# Autodesk Inventor assembly: assembled-feed
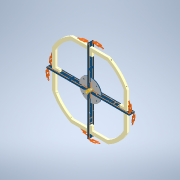
[picture p0: Inventor's stored thumbnail of the model, 180x180]
Saved by Autodesk Inventor 2021 (Build 250183000, 183)
## iProperties
Created: 2020-09-03
Part Number: assembled-feed
Document SubType Name: Assembly
Designer: dsouthall
Author: dsouthall
## iProperties of the stored document quad-slot-hub-traces.ipt
Created: 2020-10-19
Part Number: quad-slot-hub-traces
Material: Generic
Description: FreeCAD Model
Document SubType Name: Modeling
Designer: dsouthall
Authority: Unknown
Density: 1 g/cm^3
Appearance: Default
Sending System: FreeCAD
Preprocessor: Open CASCADE STEP processor 7.3
Title: C:/Users/dsouthall/OneDrive - The University of Chicago/Hpol/hpol-prototype/design/Feed Design/quad-slot-hub_revA/quad-slot-hub_revA/quad-slot-hub-traces.step
Author: Author
## iProperties of the stored document 91841A003_TYPE 18-8 STAINLESS STEEL HEX NUT.ipt
Created: 2015-02-23
Part Number: 91841A003_TYPE 18-8 STAINLESS STEEL HEX NUT
Material: Generic
Description: STEP AP203
Document SubType Name: Modeling
Designer: dsouthall
Density: 1 g/cm^3
Appearance: Default
Sending System: SolidWorks 2010
Preprocessor: SwSTEP 2.0
Title: 91841A003.step
Revision Number: ANY
## Documents named in this file (11)
- C:\Users\dsouthall\OneDrive - The University of Chicago\Hpol\hpol-prototype\design\Quad-Slot\Model 8 in\assembled-feed.iam
- C:\Users\dsouthall\OneDrive - The University of Chicago\Hpol\hpol-prototype\design\Quad-Slot\Model 8 in\assembled-feed_feedline_8in.iam
- C:\Users\dsouthall\OneDrive - The University of Chicago\Hpol\hpol-prototype\design\Quad-Slot\Model 8 in\source\standin_quad_hub.ipt
- C:\Users\dsouthall\OneDrive - The University of Chicago\Hpol\hpol-prototype\design\Quad-Slot\Model 8 in\source\insert_8in.ipt
- C:\Users\dsouthall\OneDrive - The University of Chicago\Hpol\hpol-prototype\design\Quad-Slot\Model 8 in\source\hub\COMPOUND.ipt
- **C:\Users\dsouthall\OneDrive - The University of Chicago\Hpol\hpol-prototype\design\Quad-Slot\Model 8 in\assembled-feed.iam*LocalDocs*xAaaaqbdaAaaaaaaaAaaaqho5Nc*quad-slot-hub-traces.ipt
- **C:\Users\dsouthall\OneDrive - The University of Chicago\Hpol\hpol-prototype\design\Quad-Slot\Model 8 in\assembled-feed.iam*LocalDocs*xAaaaqibaAaaaaaaaAaaaqomz3g*91841A003_TYPE 18-8 STAINLESS STEEL HEX NUT.ipt
- C:\Users\dsouthall\OneDrive - The University of Chicago\Hpol\hpol-prototype\design\Quad-Slot\Model 8 in\92196A077_18-8 STAINLESS STEEL SOCKET HEAD SCR.ipt
- C:\Users\dsouthall\OneDrive - The University of Chicago\Hpol\hpol-prototype\design\Feed Design\quad-slot-hub_revA\quad-slot-hub_revA\quad-slot-hub-traces.step
- C:\Users\dsouthall\OneDrive - The University of Chicago\Hpol\hpol-prototype\design\Quad-Slot\Model 8 in\source\91841A003_TYPE 18-8 STAINLESS STEEL HEX NUT\raw step\91841A003_TYPE 18-8 STAINLESS STEEL HEX NUT.STEP
- C:\Users\dsouthall\OneDrive - The University of Chicago\Hpol\hpol-prototype\design\Quad-Slot\Model 8 in\source\92196A077_18-8 STAINLESS STEEL SOCKET HEAD SCREW\92196A077_18-8 STAINLESS STEEL SOCKET HEAD SCREW.STEP
## Components (15 placed, 7 different names)
1. assembled-feed_feedline_8in:1 [sub-assembly] — Mate:12, Mate:13, Mate:14, Insert:1, Insert:8, Mate:20
2. assembled-feed_feedline_8in:2 [sub-assembly] — Mate:9, Mate:10, Mate:11, Mate:15, Insert:2, Insert:3
3. assembled-feed_feedline_8in:3 [sub-assembly] — Mate:6, Mate:7, Mate:8, Mate:16, Insert:4, Insert:5
4. assembled-feed_feedline_8in:4 [sub-assembly] — Mate:3, Mate:4, Mate:5, Mate:17, Insert:6, Insert:7
5. standin_quad_hub:1 — Mate:1, Mate:2, Mate:3, Mate:4, Mate:5, Mate:6, Mate:7, Mate:8, Mate:9, Mate:10, Mate:11, Mate:12, Mate:13, Mate:14, Mate:15, Mate:16, Mate:17, Mate:18, Mate:19, Angle:2, Flush:2, Mate:21
6. insert_8in:1 — Insert:1, Insert:2
7. insert_8in:2 — Insert:7, Insert:8
8. insert_8in:3 — Insert:5, Insert:6
9. insert_8in:4 — Insert:3, Insert:4
10. COMPOUND:1 — Mate:18, Mate:19, Angle:1, Insert:9, Insert:10
11. quad-slot-hub-traces:1 — Flush:2, Mate:20, Mate:21, Insert:11, Insert:12
12. 91841A003_TYPE 18-8 STAINLESS STEEL HEX NUT:1 — Insert:12
13. 91841A003_TYPE 18-8 STAINLESS STEEL HEX NUT:2 — Insert:11
14. 92196A077_18-8 STAINLESS STEEL SOCKET HEAD SCR:1 — Insert:10
15. 92196A077_18-8 STAINLESS STEEL SOCKET HEAD SCR:2 — Insert:9
## Relationships (37: Mate 21, Insert 12, Flush 2, Angle 2)
- Flush:1 (-3.9973 mm)
- Mate:1: standin_quad_hub:1
- Mate:2: standin_quad_hub:1
- Mate:3: assembled-feed_feedline_8in:4 ↔ standin_quad_hub:1
- Mate:4: assembled-feed_feedline_8in:4 ↔ standin_quad_hub:1
- Mate:5: assembled-feed_feedline_8in:4 ↔ standin_quad_hub:1
- Mate:6: assembled-feed_feedline_8in:3 ↔ standin_quad_hub:1
- Mate:7: assembled-feed_feedline_8in:3 ↔ standin_quad_hub:1
- Mate:8: assembled-feed_feedline_8in:3 ↔ standin_quad_hub:1
- Mate:9: assembled-feed_feedline_8in:2 ↔ standin_quad_hub:1
- Mate:10: assembled-feed_feedline_8in:2 ↔ standin_quad_hub:1
- Mate:11: assembled-feed_feedline_8in:2 ↔ standin_quad_hub:1
- Mate:12: assembled-feed_feedline_8in:1 ↔ standin_quad_hub:1
- Mate:13: assembled-feed_feedline_8in:1 ↔ standin_quad_hub:1
- Mate:14: assembled-feed_feedline_8in:1 ↔ standin_quad_hub:1
- Mate:15: assembled-feed_feedline_8in:2 ↔ standin_quad_hub:1
- Mate:16: assembled-feed_feedline_8in:3 ↔ standin_quad_hub:1
- Mate:17: assembled-feed_feedline_8in:4 ↔ standin_quad_hub:1
- Insert:1: assembled-feed_feedline_8in:1 ↔ insert_8in:1
- Insert:2: assembled-feed_feedline_8in:2 ↔ insert_8in:1
- Insert:3: assembled-feed_feedline_8in:2 ↔ insert_8in:4
- Insert:4: assembled-feed_feedline_8in:3 ↔ insert_8in:4
- Insert:5: assembled-feed_feedline_8in:3 ↔ insert_8in:3
- Insert:6: assembled-feed_feedline_8in:4 ↔ insert_8in:3
- Insert:7: assembled-feed_feedline_8in:4 ↔ insert_8in:2
- Insert:8: assembled-feed_feedline_8in:1 ↔ insert_8in:2
- Mate:18: standin_quad_hub:1 ↔ COMPOUND:1
- Mate:19: standin_quad_hub:1 ↔ COMPOUND:1
- Angle:1 (45 deg): COMPOUND:1
- Angle:2 (0 deg): standin_quad_hub:1
- Flush:2: standin_quad_hub:1 ↔ quad-slot-hub-traces:1
- Mate:20: assembled-feed_feedline_8in:1 ↔ quad-slot-hub-traces:1
- Mate:21: standin_quad_hub:1 ↔ quad-slot-hub-traces:1
- Insert:9: COMPOUND:1 ↔ 92196A077_18-8 STAINLESS STEEL SOCKET HEAD SCR:2
- Insert:10: COMPOUND:1 ↔ 92196A077_18-8 STAINLESS STEEL SOCKET HEAD SCR:1
- Insert:11: quad-slot-hub-traces:1 ↔ 91841A003_TYPE 18-8 STAINLESS STEEL HEX NUT:2
- Insert:12: quad-slot-hub-traces:1 ↔ 91841A003_TYPE 18-8 STAINLESS STEEL HEX NUT:1
